# Autodesk Inventor assembly: Effector
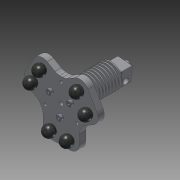
[picture p0: Inventor's stored thumbnail of the model, 180x180]
Saved by Autodesk Inventor 2014 (Build 180170000, 170)
## iProperties
Created: 2014-08-27
Part Number: Effector
Document SubType Name: Assembly
Designer: ThatOtherGuy
Author: ThatOtherGuy
## Documents named in this file (7)
- U:\Hobbies\Inventor\KosselCNC1515\Effector\Effector.iam
- U:\Hobbies\Inventor\KosselCNC1515\Effector\Effector_GrooveMount.ipt
- U:\Hobbies\Inventor\KosselCNC1515\Hotend\E3Dv5.iam
- U:\Hobbies\Inventor\KosselCNC1515\Effector\Effector_Platform_V2.ipt
- U:\Hobbies\Inventor\Content Center Files\R2014\en-US\ANSI B18.3.1M(1)\ANSI B18.3.1M - M3x0.5 x 16(2).ipt
- U:\Hobbies\Inventor\Content Center Files\R2014\en-US\ISO 10511\ISO 10511 - M3.ipt
- U:\Hobbies\Inventor\KosselCNC1515\Joints\Joint_Ball_Bearing_12MM.ipt
## Components (15 placed, 6 different names)
1. Effector_Platform:1 — Mate:8, Mate:10, Mate:11, Insert:1, Insert:3, Insert:5, Mate:12, Mate:14, Tangent:1, Tangent:2, Mate:15, Mate:16
2. Effector_GrooveMount:1 — Mate:8, Insert:6, Insert:8, Insert:10, Mate:15, Mate:16
3. E3Dv5:1 [sub-assembly] — Mate:10, Mate:11
4. Broached Socket Head Cap Screw - Metric M3x0.5 x 16:1 — Insert:1
5. Broached Socket Head Cap Screw - Metric M3x0.5 x 16:3 — Insert:3
6. Broached Socket Head Cap Screw - Metric M3x0.5 x 16:5 — Insert:5
7. DIN EN ISO 10511 M3:1 — Insert:6
8. DIN EN ISO 10511 M3:3 — Insert:8
9. DIN EN ISO 10511 M3:5 — Insert:10
10. Joint_Ball_Bearing_12MM:2 — Mate:14, Tangent:1
11. Joint_Ball_Bearing_12MM:1 — Mate:12, Tangent:2
12. Joint_Ball_Bearing_12MM:3
13. Joint_Ball_Bearing_12MM:4
14. Joint_Ball_Bearing_12MM:5
15. Joint_Ball_Bearing_12MM:6
## Component patterns: (3 elements, first: Joint_Ball_Bearing_12MM:2 + Joint_Ball_Bearing_12MM:1)
## Relationships (15: Mate 7, Insert 6, Tangent 2)
- Mate:8: Effector_Platform:1 ↔ Effector_GrooveMount:1
- Mate:10: Effector_Platform:1 ↔ E3Dv5:1
- Mate:11: Effector_Platform:1 ↔ E3Dv5:1
- Insert:1: Effector_Platform:1 ↔ Broached Socket Head Cap Screw - Metric M3x0.5 x 16:1
- Insert:3: Effector_Platform:1 ↔ Broached Socket Head Cap Screw - Metric M3x0.5 x 16:3
- Insert:5: Effector_Platform:1 ↔ Broached Socket Head Cap Screw - Metric M3x0.5 x 16:5
- Insert:6: Effector_GrooveMount:1 ↔ DIN EN ISO 10511 M3:1
- Insert:8: Effector_GrooveMount:1 ↔ DIN EN ISO 10511 M3:3
- Insert:10: Effector_GrooveMount:1 ↔ DIN EN ISO 10511 M3:5
- Mate:12: Effector_Platform:1 ↔ Joint_Ball_Bearing_12MM:1
- Mate:14: Effector_Platform:1 ↔ Joint_Ball_Bearing_12MM:2
- Tangent:1 (-2.35 mm): Effector_Platform:1 ↔ Joint_Ball_Bearing_12MM:2
- Tangent:2 (-2.35 mm): Effector_Platform:1 ↔ Joint_Ball_Bearing_12MM:1
- Mate:15: Effector_Platform:1 ↔ Effector_GrooveMount:1
- Mate:16: Effector_Platform:1 ↔ Effector_GrooveMount:1
